# Autodesk Inventor assembly: Level 1 Frame
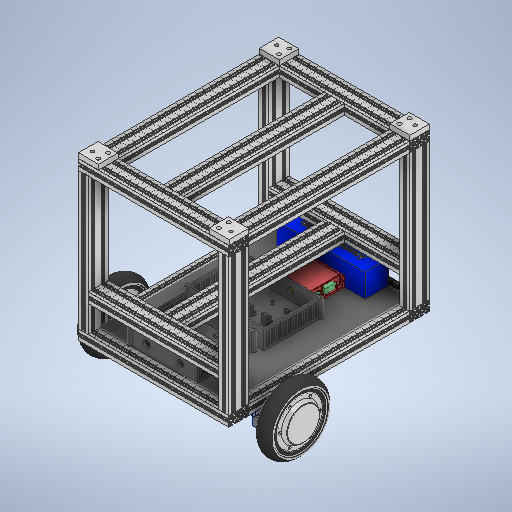
[picture p0: Inventor's stored thumbnail of the model, 512x512]
Saved by Autodesk Inventor 2026.2 (Build 302298010, 298A)
## iProperties
Created: 2026-03-27
Part Number: Level 1 Frame
Document SubType Name: Assembly
Designer: chanh
Author: chanh
## Documents named in this file (17)
- C:\Users\chanh\내 드라이브\교과공부\2026년 1학기 (4학년 1학기)\01창의제품설계\CLOSE_hardware\02하체\도면\Level 1 Frame.iam
- C:\Users\chanh\내 드라이브\교과공부\2026년 1학기 (4학년 1학기)\01창의제품설계\CLOSE_hardware\02하체\3060 Aluminium Profile 450mm.ipt
- C:\Users\chanh\내 드라이브\교과공부\2026년 1학기 (4학년 1학기)\01창의제품설계\CLOSE_hardware\02하체\3060 Aluminium Profile 480mm.ipt
- C:\Users\chanh\내 드라이브\교과공부\2026년 1학기 (4학년 1학기)\01창의제품설계\CLOSE_hardware\00부품\ZLLG80ASM250-L V3.0 (모터)\ZLLG80ASM250-L V3.0 Single shaft.iam
- C:\Users\chanh\내 드라이브\교과공부\2026년 1학기 (4학년 1학기)\01창의제품설계\CLOSE_hardware\00부품\ZLAC8015D V4.0 (드라이버)\ZLAC8015D V4.0.iam
- C:\Users\chanh\내 드라이브\교과공부\2026년 1학기 (4학년 1학기)\01창의제품설계\CLOSE_hardware\00부품\ZLLG80ASM250-L V3.0 (모터)\Nut.ipt
- C:\Users\chanh\내 드라이브\교과공부\2026년 1학기 (4학년 1학기)\01창의제품설계\CLOSE_hardware\02하체\motor_bracket.ipt
- C:\Users\chanh\내 드라이브\교과공부\2026년 1학기 (4학년 1학기)\01창의제품설계\CLOSE_hardware\02하체\Bottom_Plate_Acryl.ipt
- C:\Users\chanh\내 드라이브\교과공부\2026년 1학기 (4학년 1학기)\01창의제품설계\CLOSE_hardware\02하체\Battery.ipt
- C:\Users\chanh\내 드라이브\교과공부\2026년 1학기 (4학년 1학기)\01창의제품설계\CLOSE_hardware\02하체\assist_wheel.iam
- C:\Users\chanh\내 드라이브\교과공부\2026년 1학기 (4학년 1학기)\01창의제품설계\CLOSE_hardware\02하체\assist_wheel_bracket.ipt
- C:\Users\chanh\내 드라이브\교과공부\2026년 1학기 (4학년 1학기)\01창의제품설계\CLOSE_hardware\02하체\3060 Aluminium Profile 410mm.ipt
- C:\Users\chanh\내 드라이브\교과공부\2026년 1학기 (4학년 1학기)\01창의제품설계\CLOSE_hardware\02하체\3060 Aluminium Profile 390mm.ipt
- C:\Users\chanh\내 드라이브\교과공부\2026년 1학기 (4학년 1학기)\01창의제품설계\CLOSE_hardware\02하체\Lift Bracket other side.ipt
- C:\Users\chanh\내 드라이브\교과공부\2026년 1학기 (4학년 1학기)\01창의제품설계\CLOSE_hardware\02하체\Lift Bracket.ipt
- C:\Users\chanh\내 드라이브\교과공부\2026년 1학기 (4학년 1학기)\01창의제품설계\CLOSE_hardware\02하체\Power Box (12V).ipt
- C:\Users\chanh\내 드라이브\교과공부\2026년 1학기 (4학년 1학기)\01창의제품설계\CLOSE_hardware\02하체\Power Box (24V).ipt
## Components (34 placed, 16 different names)
1. Lift Bracket:2 — Flush:59, Flush:60, Mate:40
2. Lift Bracket:1 — Flush:57, Mate:39, Flush:58
3. Lift Bracket other side:2 — Mate:42, Flush:63, Flush:64
4. Lift Bracket other side:1 — Mate:41, Flush:61, Flush:62
5. 3060 Aluminium Profile 480mm:1 — Mate:2, Flush:6, Flush:7, Mate:4, Flush:8, Flush:9, Flush:10, Flush:17, Mate:15
6. 3060 Aluminium Profile 480mm:2 — Mate:3, Flush:4, Flush:5, Flush:11, Mate:13, Mate:14
7. 3060 Aluminium Profile 480mm:3 — Flush:13, Mate:8, Flush:14, Mate:9
8. 3060 Aluminium Profile 480mm:4 — Flush:31, Mate:25, Flush:38
9. 3060 Aluminium Profile 480mm:5 — Flush:30, Mate:24, Flush:37
10. 3060 Aluminium Profile 480mm:6 — Flush:32, Mate:26, Flush:39
11. 3060 Aluminium Profile 480mm:7 — Mate:30, Flush:43, Flush:44
12. 3060 Aluminium Profile 450mm:1 — Flush:2, Mate:1, Flush:3, Mate:2, Mate:3, Flush:4, Flush:5, Flush:6, Flush:7, Mate:18, Mate:21, Flush:24, Flush:25, Flush:26, Flush:27
13. 3060 Aluminium Profile 450mm:2 — Mate:4, Flush:8, Flush:9, Flush:13, Mate:8, Mate:16, Flush:18, Mate:20, Flush:22, Flush:23, Mate:19, Flush:28, Flush:29, Mate:28
14. 3060 Aluminium Profile 450mm:3 — Mate:22, Flush:35, Flush:36, Mate:24, Flush:37, Mate:25, Flush:38, Mate:26, Flush:57, Mate:39, Flush:58, Mate:42, Flush:63, Flush:64
15. 3060 Aluminium Profile 450mm:4 — Mate:23, Flush:30, Flush:31, Flush:32, Flush:33, Flush:34, Flush:39, Flush:59, Flush:60, Mate:40, Mate:41, Flush:61, Flush:62
16. 3060 Aluminium Profile 410mm:1 — Mate:19, Flush:28, Flush:29, Mate:22, Mate:27, Flush:40
17. 3060 Aluminium Profile 410mm:2 — Mate:18, Flush:26, Flush:27, Mate:23, Mate:29, Flush:41
18. 3060 Aluminium Profile 410mm:3 — Mate:21, Flush:24, Flush:25, Flush:33, Flush:34
19. 3060 Aluminium Profile 410mm:4 — Mate:20, Flush:22, Flush:23, Flush:35, Flush:36
20. 3060 Aluminium Profile 390mm:1 — Mate:29, Flush:41, Flush:42, Flush:43
21. 3060 Aluminium Profile 390mm:2 — Mate:27, Flush:40, Mate:28, Flush:42, Mate:30, Flush:44
22. ZLLG80ASM250-L V3.0 Single shaft:1 [sub-assembly] — Rigid:3
23. ZLLG80ASM250-L V3.0 Single shaft:2 [sub-assembly] — Rigid:1
24. ZLAC8015D V4.0:1 [sub-assembly] — Mate:10, Mate:74, Flush:75
25. Nut:1 — Rigid:2
26. Nut:2 — Rigid:4
27. motor_bracket:1 — Flush:10, Flush:17, Rigid:1, Rigid:2, Mate:15
28. motor_bracket:2 — Flush:11, Mate:13, Rigid:3, Rigid:4, Mate:14
29. assist_wheel:1 [sub-assembly] — Tangent:1, Mate:17, Flush:20, Flush:21
30. assist_wheel_bracket:1 — Mate:16, Flush:18, Flush:19, Mate:17, Flush:20
31. Power Box (24V):1 — Mate:79, Mate:80, Mate:81
32. Power Box (12V):1 — Mate:75, Flush:76, Mate:78, Mate:80
33. Battery:1 — Mate:11, Flush:73, Flush:74, Mate:74
34. Bottom_Plate_Acryl:1 — Mate:9, Flush:15, Flush:16, Mate:10, Mate:11, Angle:1, Flush:74, Mate:75, Flush:76, Mate:79
## Relationships (97: Flush 55, Mate 36, WeldJoint 4, Angle 1, Tangent 1)
- Flush:1 (-240 mm)
- Flush:2: 3060 Aluminium Profile 450mm:1
- Mate:1: 3060 Aluminium Profile 450mm:1
- Flush:3: 3060 Aluminium Profile 450mm:1
- Mate:2: 3060 Aluminium Profile 480mm:1 ↔ 3060 Aluminium Profile 450mm:1
- Mate:3: 3060 Aluminium Profile 480mm:2 ↔ 3060 Aluminium Profile 450mm:1
- Flush:4: 3060 Aluminium Profile 480mm:2 ↔ 3060 Aluminium Profile 450mm:1
- Flush:5: 3060 Aluminium Profile 480mm:2 ↔ 3060 Aluminium Profile 450mm:1
- Flush:6: 3060 Aluminium Profile 480mm:1 ↔ 3060 Aluminium Profile 450mm:1
- Flush:7: 3060 Aluminium Profile 480mm:1 ↔ 3060 Aluminium Profile 450mm:1
- Mate:4: 3060 Aluminium Profile 480mm:1 ↔ 3060 Aluminium Profile 450mm:2
- Flush:8: 3060 Aluminium Profile 480mm:1 ↔ 3060 Aluminium Profile 450mm:2
- Flush:9: 3060 Aluminium Profile 480mm:1 ↔ 3060 Aluminium Profile 450mm:2
- Flush:10: 3060 Aluminium Profile 480mm:1 ↔ motor_bracket:1
- Flush:17 (150 mm): 3060 Aluminium Profile 480mm:1 ↔ motor_bracket:1
- Rigid:1 [WeldJoint]: ZLLG80ASM250-L V3.0 Single shaft:2 ↔ motor_bracket:1
- Rigid:2 [WeldJoint]: Nut:1 ↔ motor_bracket:1
- Flush:11: 3060 Aluminium Profile 480mm:2 ↔ motor_bracket:2
- Mate:13 (-150 mm): 3060 Aluminium Profile 480mm:2 ↔ motor_bracket:2
- Rigid:3 [WeldJoint]: ZLLG80ASM250-L V3.0 Single shaft:1 ↔ motor_bracket:2
- Rigid:4 [WeldJoint]: Nut:2 ↔ motor_bracket:2
- Flush:13: 3060 Aluminium Profile 480mm:3 ↔ 3060 Aluminium Profile 450mm:2
- Mate:8: 3060 Aluminium Profile 480mm:3 ↔ 3060 Aluminium Profile 450mm:2
- Flush:14: 3060 Aluminium Profile 480mm:3
- Mate:9: 3060 Aluminium Profile 480mm:3 ↔ Bottom_Plate_Acryl:1
- Flush:15: Bottom_Plate_Acryl:1
- Flush:16: Bottom_Plate_Acryl:1
- Mate:10: ZLAC8015D V4.0:1 ↔ Bottom_Plate_Acryl:1
- Mate:11: Battery:1 ↔ Bottom_Plate_Acryl:1
- Mate:14: 3060 Aluminium Profile 480mm:2 ↔ motor_bracket:2
- Mate:15: 3060 Aluminium Profile 480mm:1 ↔ motor_bracket:1
- Angle:1 (0 deg): Bottom_Plate_Acryl:1
- Tangent:1: assist_wheel:1
- Mate:16: 3060 Aluminium Profile 450mm:2 ↔ assist_wheel_bracket:1
- Flush:18: 3060 Aluminium Profile 450mm:2 ↔ assist_wheel_bracket:1
- Flush:19: assist_wheel_bracket:1
- Mate:17: assist_wheel:1 ↔ assist_wheel_bracket:1
- Flush:20: assist_wheel:1 ↔ assist_wheel_bracket:1
- Flush:21: assist_wheel:1
- Mate:18: 3060 Aluminium Profile 450mm:1 ↔ 3060 Aluminium Profile 410mm:2
- Mate:19: 3060 Aluminium Profile 450mm:2 ↔ 3060 Aluminium Profile 410mm:1
- Mate:20: 3060 Aluminium Profile 450mm:2 ↔ 3060 Aluminium Profile 410mm:4
- Mate:21: 3060 Aluminium Profile 450mm:1 ↔ 3060 Aluminium Profile 410mm:3
- Flush:22: 3060 Aluminium Profile 450mm:2 ↔ 3060 Aluminium Profile 410mm:4
- Flush:23: 3060 Aluminium Profile 450mm:2 ↔ 3060 Aluminium Profile 410mm:4
- Flush:24: 3060 Aluminium Profile 450mm:1 ↔ 3060 Aluminium Profile 410mm:3
- Flush:25: 3060 Aluminium Profile 450mm:1 ↔ 3060 Aluminium Profile 410mm:3
- Flush:26: 3060 Aluminium Profile 450mm:1 ↔ 3060 Aluminium Profile 410mm:2
- Flush:27: 3060 Aluminium Profile 450mm:1 ↔ 3060 Aluminium Profile 410mm:2
- Flush:28: 3060 Aluminium Profile 450mm:2 ↔ 3060 Aluminium Profile 410mm:1
- Flush:29: 3060 Aluminium Profile 450mm:2 ↔ 3060 Aluminium Profile 410mm:1
- Mate:22: 3060 Aluminium Profile 450mm:3 ↔ 3060 Aluminium Profile 410mm:1
- Mate:23: 3060 Aluminium Profile 450mm:4 ↔ 3060 Aluminium Profile 410mm:2
- Flush:30: 3060 Aluminium Profile 480mm:5 ↔ 3060 Aluminium Profile 450mm:4
- Flush:31: 3060 Aluminium Profile 480mm:4 ↔ 3060 Aluminium Profile 450mm:4
- Flush:32: 3060 Aluminium Profile 480mm:6 ↔ 3060 Aluminium Profile 450mm:4
- Flush:33: 3060 Aluminium Profile 450mm:4 ↔ 3060 Aluminium Profile 410mm:3
- Flush:34: 3060 Aluminium Profile 450mm:4 ↔ 3060 Aluminium Profile 410mm:3
- Flush:35: 3060 Aluminium Profile 450mm:3 ↔ 3060 Aluminium Profile 410mm:4
- Flush:36: 3060 Aluminium Profile 450mm:3 ↔ 3060 Aluminium Profile 410mm:4
- Mate:24: 3060 Aluminium Profile 480mm:5 ↔ 3060 Aluminium Profile 450mm:3
- Flush:37: 3060 Aluminium Profile 480mm:5 ↔ 3060 Aluminium Profile 450mm:3
- Mate:25: 3060 Aluminium Profile 480mm:4 ↔ 3060 Aluminium Profile 450mm:3
- Flush:38: 3060 Aluminium Profile 480mm:4 ↔ 3060 Aluminium Profile 450mm:3
- Mate:26: 3060 Aluminium Profile 480mm:6 ↔ 3060 Aluminium Profile 450mm:3
- Flush:39: 3060 Aluminium Profile 480mm:6 ↔ 3060 Aluminium Profile 450mm:4
- Mate:27: 3060 Aluminium Profile 410mm:1 ↔ 3060 Aluminium Profile 390mm:2
- Flush:40: 3060 Aluminium Profile 410mm:1 ↔ 3060 Aluminium Profile 390mm:2
- Mate:28 (80 mm): 3060 Aluminium Profile 450mm:2 ↔ 3060 Aluminium Profile 390mm:2
- Mate:29: 3060 Aluminium Profile 410mm:2 ↔ 3060 Aluminium Profile 390mm:1
- Flush:41: 3060 Aluminium Profile 410mm:2 ↔ 3060 Aluminium Profile 390mm:1
- Flush:42: 3060 Aluminium Profile 390mm:1 ↔ 3060 Aluminium Profile 390mm:2
- Mate:30: 3060 Aluminium Profile 480mm:7 ↔ 3060 Aluminium Profile 390mm:2
- Flush:43: 3060 Aluminium Profile 480mm:7 ↔ 3060 Aluminium Profile 390mm:1
- Flush:44: 3060 Aluminium Profile 480mm:7 ↔ 3060 Aluminium Profile 390mm:2
- Flush:57: Lift Bracket:1 ↔ 3060 Aluminium Profile 450mm:3
- Mate:39: Lift Bracket:1 ↔ 3060 Aluminium Profile 450mm:3
- Flush:58 (1 mm): Lift Bracket:1 ↔ 3060 Aluminium Profile 450mm:3
- Flush:59: Lift Bracket:2 ↔ 3060 Aluminium Profile 450mm:4
- Flush:60 (1 mm): Lift Bracket:2 ↔ 3060 Aluminium Profile 450mm:4
- Mate:40: Lift Bracket:2 ↔ 3060 Aluminium Profile 450mm:4
- Mate:41: Lift Bracket other side:1 ↔ 3060 Aluminium Profile 450mm:4
- Flush:61 (1 mm): Lift Bracket other side:1 ↔ 3060 Aluminium Profile 450mm:4
- Flush:62: Lift Bracket other side:1 ↔ 3060 Aluminium Profile 450mm:4
- Mate:42: Lift Bracket other side:2 ↔ 3060 Aluminium Profile 450mm:3
- Flush:63: Lift Bracket other side:2 ↔ 3060 Aluminium Profile 450mm:3
- Flush:64 (1 mm): Lift Bracket other side:2 ↔ 3060 Aluminium Profile 450mm:3
- Flush:73: Battery:1
- Flush:74: Battery:1 ↔ Bottom_Plate_Acryl:1
- Mate:74: ZLAC8015D V4.0:1 ↔ Battery:1
- Flush:75: ZLAC8015D V4.0:1
- Mate:75: Power Box (12V):1 ↔ Bottom_Plate_Acryl:1
- Flush:76: Power Box (12V):1 ↔ Bottom_Plate_Acryl:1
- Mate:78: Power Box (12V):1
- Mate:79: Power Box (24V):1 ↔ Bottom_Plate_Acryl:1
- Mate:80 (15 mm): Power Box (24V):1 ↔ Power Box (12V):1
- Mate:81: Power Box (24V):1
